# Autodesk Inventor assembly: highlevel
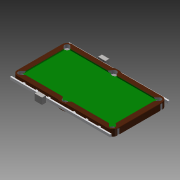
[picture p0: Inventor's stored thumbnail of the model, 180x180]
Saved by Autodesk Inventor 2015 (Build 190159000, 159)
## iProperties
Created: 2016-12-01
Part Number: highlevel
Document SubType Name: Assembly
Designer: Ernest
Author: Ernest
## Documents named in this file (4)
- C:\Users\Ernest\Documents\Capstone-Project\doc\CAD\HighLevel\highlevel.iam
- C:\Users\Ernest\Documents\Capstone-Project\doc\CAD\Pool Table\Table_Model.ipt
- C:\Users\Ernest\Documents\Capstone-Project\doc\CAD\HighLevel\Rail.ipt
- C:\Users\Ernest\Documents\Capstone-Project\doc\CAD\HighLevel\ArmBase3.ipt
## Components (5 placed, 3 different names)
1. Table_Model:1 — Mate:1, Flush:1, Mate:2, Flush:4, Flush:7
2. Rail:1 — Mate:1, Flush:1, Flush:2, Flush:3, Flush:4, Mate:4
3. Rail:2 — Flush:2, Flush:3, Mate:2, Mate:3
4. ArmBase3:1 — Flush:5, Flush:6, Mate:4, Flush:7
5. ArmBase3:2 — Flush:5, Flush:6, Mate:3
## Relationships (11: Flush 7, Mate 4)
- Mate:1: Table_Model:1 ↔ Rail:1
- Flush:1: Table_Model:1 ↔ Rail:1
- Flush:2: Rail:1 ↔ Rail:2
- Flush:3: Rail:1 ↔ Rail:2
- Mate:2: Table_Model:1 ↔ Rail:2
- Flush:4 (42.261 mm): Table_Model:1 ↔ Rail:1
- Flush:5: ArmBase3:1 ↔ ArmBase3:2
- Flush:6: ArmBase3:1 ↔ ArmBase3:2
- Mate:3: Rail:2 ↔ ArmBase3:2
- Mate:4: Rail:1 ↔ ArmBase3:1
- Flush:7: Table_Model:1 ↔ ArmBase3:1
